# Autodesk Inventor assembly: ServoWithShaftAssembly
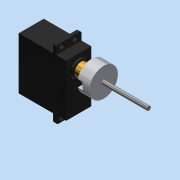
[picture p0: Inventor's stored thumbnail of the model, 180x180]
Saved by Autodesk Inventor 2017 (Build 210142000, 142)
## iProperties
Created: 2016-11-03
Part Number: ServoWithShaftAssembly
Document SubType Name: Assembly
Designer: techn
Author: techn
## Documents named in this file (5)
- E:\OneDrive\Documents\Other Projects\Submarine\CAD\common\3mmShaftToServo\ServoWithShaftAssembly.iam
- E:\OneDrive\Documents\Other Projects\Submarine\CAD\common\HitecServo\HitecServoAssembly.iam
- E:\OneDrive\Documents\Other Projects\Submarine\CAD\common\3mmShaftToServo\.125InchServoDrivenShaft.ipt
- E:\OneDrive\Documents\Other Projects\Submarine\CAD\midships\AftServoSection\ServoShaftCoupler\ServoShaftCouplerAssembly.iam
- E:\OneDrive\Documents\Other Projects\Submarine\CAD\midships\AftServoSection\ServoShaftCoupler\EncoderDisc.ipt
## Components (4 placed, 4 different names)
1. HitecServoAssembly:1 [sub-assembly] — Mate:1, Mate:2, Angle:1, Angle:2
2. ServoShaftCouplerAssembly:1 [sub-assembly] — Mate:1, Mate:2, Mate:3, Mate:4, Angle:1, Mate:6
3. .125InchServoDrivenShaft:1 — Mate:3, Mate:4, Mate:5
4. EncoderDisc:1 — Mate:5, Mate:6, Angle:2
## Relationships (8: Mate 6, Angle 2)
- Mate:1: HitecServoAssembly:1 ↔ ServoShaftCouplerAssembly:1
- Mate:2 (0.254 mm): HitecServoAssembly:1 ↔ ServoShaftCouplerAssembly:1
- Mate:3: ServoShaftCouplerAssembly:1 ↔ .125InchServoDrivenShaft:1
- Mate:4 (0.508 mm): ServoShaftCouplerAssembly:1 ↔ .125InchServoDrivenShaft:1
- Angle:1 (0 deg): HitecServoAssembly:1 ↔ ServoShaftCouplerAssembly:1
- Mate:5: .125InchServoDrivenShaft:1 ↔ EncoderDisc:1
- Mate:6: ServoShaftCouplerAssembly:1 ↔ EncoderDisc:1
- Angle:2 (90 deg): HitecServoAssembly:1 ↔ EncoderDisc:1
